# Autodesk Inventor assembly: outer_cover
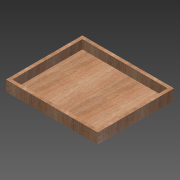
[picture p0: Inventor's stored thumbnail of the model, 180x180]
Saved by Autodesk Inventor 2014 SP1 (Build 180222100, 222)
## iProperties
Created: 2014-02-23
Part Number: outer_cover
Document SubType Name: Assembly
Designer: Chris
Mass: 4427 g
Surface Area: 8325.18 cm^2
Volume: 4427 cm^3
Density: 1 g/cm^3
Author: Chris
## Documents named in this file (4)
- C:\Users\Chris\Documents\projects\langstroth_plain\outer_cover\outer_cover.iam
- C:\Users\Chris\Documents\projects\langstroth_plain\outer_cover\outer_cover_sheet.ipt
- C:\Users\Chris\Documents\projects\langstroth_plain\outer_cover\outer_cover_side.ipt
- C:\Users\Chris\Documents\projects\langstroth_plain\outer_cover\outer_cover_end.ipt
## Components (5 placed, 3 different names)
1. outer_cover_sheet:1 — Mate:1, Mate:2, Mate:3, Mate:4, Mate:5
2. outer_cover_side:1 — Flush:2, Mate:4, Flush:4, Flush:5
3. outer_cover_side:2 — Flush:1, Flush:2, Mate:3, Flush:6, Flush:7
4. outer_cover_end:1 — Flush:3, Mate:5, Flush:5, Flush:6
5. outer_cover_end:2 — Flush:1, Flush:3, Mate:1, Mate:2, Flush:4, Flush:7
## Relationships (12: Flush 7, Mate 5)
- Flush:1: outer_cover_side:2 ↔ outer_cover_end:2
- Flush:2: outer_cover_side:1 ↔ outer_cover_side:2
- Flush:3: outer_cover_end:1 ↔ outer_cover_end:2
- Mate:1: outer_cover_sheet:1 ↔ outer_cover_end:2
- Mate:2: outer_cover_sheet:1 ↔ outer_cover_end:2
- Mate:3: outer_cover_sheet:1 ↔ outer_cover_side:2
- Mate:4: outer_cover_sheet:1 ↔ outer_cover_side:1
- Mate:5: outer_cover_sheet:1 ↔ outer_cover_end:1
- Flush:4: outer_cover_side:1 ↔ outer_cover_end:2
- Flush:5: outer_cover_side:1 ↔ outer_cover_end:1
- Flush:6: outer_cover_side:2 ↔ outer_cover_end:1
- Flush:7: outer_cover_side:2 ↔ outer_cover_end:2
